# Autodesk Inventor assembly: Wrist2
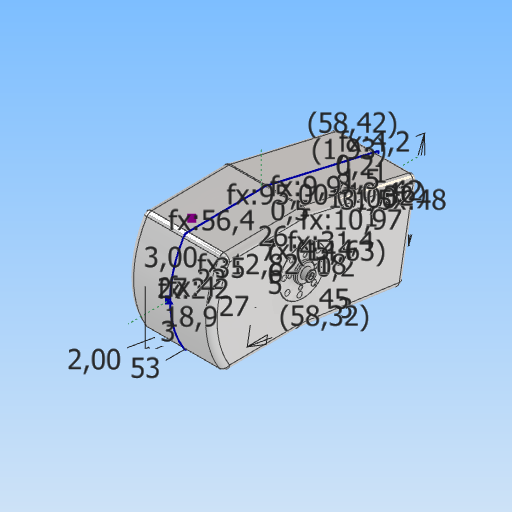
[picture p0: Inventor's stored thumbnail of the model, 512x512]
Saved by Autodesk Inventor 2020.2 (Build 242310000, 310)
## iProperties
Created: 2020-02-07
Part Number: Wrist2
Document SubType Name: Assembly
Designer: JochenAlt
Author: JochenAlt
## Documents named in this file (9)
- D:\Projects\MiniBot\CAD\Wrist.iam
- D:\Projects\MiniBot\CAD\extern\Herkulex\Herkulex DRS-040x.ipt
- D:\Projects\MiniBot\CAD\extern\Herkulex\Herkulex DRS-020x.ipt
- D:\Projects\MiniBot\CAD\extern\bearings\20x27x4\W 61704-2ZS.iam
- D:\Projects\MiniBot\CAD\extern\bearings\25x32x4\W 61705-2RS1.iam
- D:\Projects\MiniBot\CAD\Wrist.ipt
- D:\Projects\MiniBot\CAD\WristFlange.ipt
- D:\Projects\MiniBot\CAD\gripper\Base\Konstruktions-Assistent\Stirnzahnrad23.ipt
- D:\Projects\MiniBot\CAD\dimensions.xlsx
## Components (8 placed, 7 different names)
1. Herkulex DRS-0201:1 — Passend:28, Passend:30, Passend:42, Winkel:2, Passend:43, Passend:44, Passend:45
2. Herkulex DRS-040x:1 — Passend:36, Fluchtend:1, Winkel:1
3. W 61704-2ZS:2 [sub-assembly]
4. W 61705-2RS1:1 [sub-assembly] — Passend:32, Passend:37, Passend:46, Passend:47
5. Wrist:1 — Passend:32, Passend:33, Passend:34, Passend:36, Fluchtend:1, Winkel:1, Passend:37, Passend:42, Passend:43
6. W 61705-2RS1:2 [sub-assembly] — Passend:33, Passend:34
7. WristFlange:1 — Passend:46, Passend:47
8. Stirnzahnrad2:1 — Passend:44, Passend:45
## Relationships (16: Mate 13, Angle 2, Flush 1)
- Passend:28 [Mate]: Herkulex DRS-0201:1
- Passend:30 [Mate]: Herkulex DRS-0201:1
- Passend:32 [Mate]: W 61705-2RS1:1 ↔ Wrist:1
- Passend:33 [Mate]: Wrist:1 ↔ W 61705-2RS1:2
- Passend:34 [Mate]: Wrist:1 ↔ W 61705-2RS1:2
- Passend:36 [Mate]: Herkulex DRS-040x:1 ↔ Wrist:1
- Fluchtend:1 [Flush]: Herkulex DRS-040x:1 ↔ Wrist:1
- Winkel:1 [Angle] (180 deg): Herkulex DRS-040x:1 ↔ Wrist:1
- Passend:37 [Mate] (0.1 mm): W 61705-2RS1:1 ↔ Wrist:1
- Passend:42 [Mate]: Herkulex DRS-0201:1 ↔ Wrist:1
- Winkel:2 [Angle] (180 deg): Herkulex DRS-0201:1
- Passend:43 [Mate] (0.2 mm): Herkulex DRS-0201:1 ↔ Wrist:1
- Passend:44 [Mate]: Herkulex DRS-0201:1 ↔ Stirnzahnrad2:1
- Passend:45 [Mate]: Herkulex DRS-0201:1 ↔ Stirnzahnrad2:1
- Passend:46 [Mate]: W 61705-2RS1:1 ↔ WristFlange:1
- Passend:47 [Mate]: W 61705-2RS1:1 ↔ WristFlange:1
## Named parameters: roundness_small = 3 mm, roundness_tiny = 0.5 mm, wall_thickness = 3 mm, medium_arm_width = 51 mm, big_arm_width = 56 mm, bevel_angle = 20 deg, medium_arm_radius = 35 mm, big_arm_radius = 48 mm, medium_arm_circle_centre = 11 mm, big_arm_circle_centre = 25 mm, thickness = 3 mm, tight_fit = 0.2 mm, press_fit = 0.1 mm, m2_screw_hole_diameter = 2.2 mm, m2_hex_width = 4.2 mm, m2_washer_diameter = 5.2 mm, m2_allen_screw_width = 4 mm, m2_allen_screw_height = 2 mm, m2_washer_height = 0.3 mm
